# Autodesk Inventor assembly: Assembly2
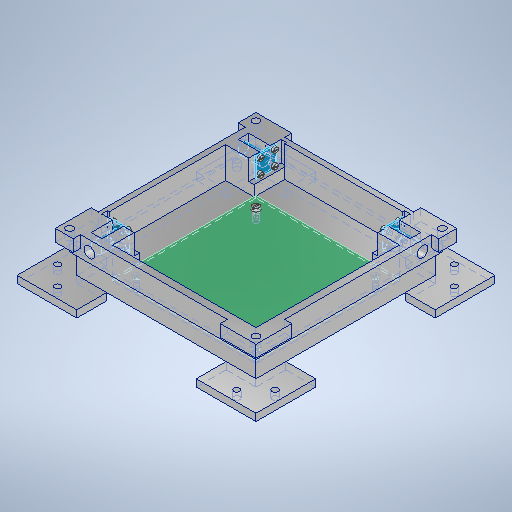
[picture p0: Inventor's stored thumbnail of the model, 512x512]
Saved by Autodesk Inventor 2025 (Build 290162000, 162)
## iProperties
Created: 2024-04-12
Part Number: Assembly2
Document SubType Name: Assembly
Designer: mahal
Author: mahal
## Documents named in this file (6)
- A:\study\IIST  COURSE\4th sem\MACHINING\project\Assembly2.iam
- A:\study\IIST  COURSE\4th sem\MACHINING\project\lower half.ipt
- A:\study\IIST  COURSE\4th sem\MACHINING\project\PCB.ipt
- A:\study\IIST  COURSE\4th sem\MACHINING\project\BNC connector.ipt
- C:\Users\mahal\OneDrive\Documents\Inventor\Content Center Files\R2025\en-US\UNI 6107\UNI 6107 - M3.5 x  5.ipt
- C:\Users\mahal\OneDrive\Documents\Inventor\Content Center Files\R2025\en-US\UNI 6107\UNI 6107 - M2.5 x  3.ipt
## Components (21 placed, 5 different names)
1. lower half:1 — Insert:1, Insert:2, Insert:3, Insert:4
2. PCB:1 — Insert:1, Insert:5, Insert:6, Insert:7, Insert:8
3. BNC connector:1 — Insert:3, Insert:17, Insert:18, Insert:19, Insert:20
4. BNC connector:2 — Insert:2, Insert:13, Insert:14, Insert:15, Insert:16
5. BNC connector:3 — Insert:4, Insert:9, Insert:10, Insert:11, Insert:12
6. UNI 6107 M3.5 x  5:1 — Insert:5
7. UNI 6107 M3.5 x  5:2 — Insert:6
8. UNI 6107 M3.5 x  5:3 — Insert:7
9. UNI 6107 M3.5 x  5:4 — Insert:8
10. UNI 6107 M2.5 x  3:1 — Insert:9
11. UNI 6107 M2.5 x  3:2 — Insert:10
12. UNI 6107 M2.5 x  3:3 — Insert:11
13. UNI 6107 M2.5 x  3:4 — Insert:12
14. UNI 6107 M2.5 x  3:5 — Insert:13
15. UNI 6107 M2.5 x  3:6 — Insert:14
16. UNI 6107 M2.5 x  3:7 — Insert:15
17. UNI 6107 M2.5 x  3:8 — Insert:16
18. UNI 6107 M2.5 x  3:9 — Insert:17
19. UNI 6107 M2.5 x  3:10 — Insert:18
20. UNI 6107 M2.5 x  3:11 — Insert:19
21. UNI 6107 M2.5 x  3:12 — Insert:20
## Relationships (20: Insert 20)
- Insert:1: lower half:1 ↔ PCB:1
- Insert:2: lower half:1 ↔ BNC connector:2
- Insert:3: lower half:1 ↔ BNC connector:1
- Insert:4: lower half:1 ↔ BNC connector:3
- Insert:5: PCB:1 ↔ UNI 6107 M3.5 x  5:1
- Insert:6: PCB:1 ↔ UNI 6107 M3.5 x  5:2
- Insert:7: PCB:1 ↔ UNI 6107 M3.5 x  5:3
- Insert:8: PCB:1 ↔ UNI 6107 M3.5 x  5:4
- Insert:9: BNC connector:3 ↔ UNI 6107 M2.5 x  3:1
- Insert:10: BNC connector:3 ↔ UNI 6107 M2.5 x  3:2
- Insert:11: BNC connector:3 ↔ UNI 6107 M2.5 x  3:3
- Insert:12: BNC connector:3 ↔ UNI 6107 M2.5 x  3:4
- Insert:13: BNC connector:2 ↔ UNI 6107 M2.5 x  3:5
- Insert:14: BNC connector:2 ↔ UNI 6107 M2.5 x  3:6
- Insert:15: BNC connector:2 ↔ UNI 6107 M2.5 x  3:7
- Insert:16: BNC connector:2 ↔ UNI 6107 M2.5 x  3:8
- Insert:17: BNC connector:1 ↔ UNI 6107 M2.5 x  3:9
- Insert:18: BNC connector:1 ↔ UNI 6107 M2.5 x  3:10
- Insert:19: BNC connector:1 ↔ UNI 6107 M2.5 x  3:11
- Insert:20: BNC connector:1 ↔ UNI 6107 M2.5 x  3:12
